# Autodesk Inventor assembly: Assembly1
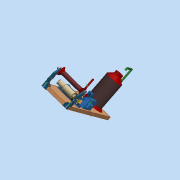
[picture p0: Inventor's stored thumbnail of the model, 180x180]
Saved by Autodesk Inventor 2019 (Build 230136000, 136)
## iProperties
Part Number: Assembly1
Document SubType Name: Assembly
Designer: Dell
Author: Dell
## Documents named in this file (18)
- C:\Users\Dell\Documents\exploration\Assembly1.iam
- C:\Users\Dell\Documents\exploration\base.ipt
- C:\Users\Dell\Documents\exploration\part1.ipt
- C:\Users\Dell\Documents\exploration\part1_MIR.ipt
- C:\Users\Dell\Documents\exploration\part5.ipt
- C:\Users\Dell\Documents\exploration\part3.ipt
- C:\Users\Dell\Documents\exploration\part7.ipt
- C:\Users\Dell\Documents\exploration\spool 2.ipt
- C:\Users\Dell\Documents\Inventor\Content Center Files\R2019\en-US\UNI ISO 1224 M\ISO 1224 - 18 4 x  9 x  2.5.ipt
- C:\Users\Dell\Documents\exploration\spool part.ipt
- C:\Users\Dell\Documents\exploration\spool new.ipt
- C:\Users\Dell\Documents\Inventor\Content Center Files\R2019\en-US\GB 29.2-88\Bolt GB 29.2 M4 x 8.ipt
- C:\Users\Dell\Documents\exploration\hook stand new.ipt
- C:\Users\Dell\Documents\exploration\belt drive part 1.ipt
- C:\Users\Dell\Documents\exploration\dc motor.ipt
- C:\Users\Dell\Documents\exploration\belt drive part 2.ipt
- C:\Users\Dell\Documents\exploration\Part4.ipt
- C:\Users\Dell\Documents\exploration\servo motor.ipt
## Components (21 placed, 17 different names)
1. base:1 — Rotational:1, Rotational:2, Rigid:1, Rigid:2, Rotational:3, Rotational:4, Rigid:6
2. part1:1 — Rotational:1, Cylindrical:1, Rotational:5, Rigid:7
3. part1_MIR:1 — Rotational:2, Rigid:3, Rigid:5
4. part5:1 — Rigid:1, Rigid:9, Rotational:7, Rotational:8
5. part3:1 — Rigid:2
6. part7:1 — Rotational:3
7. spool 2:1 — Rotational:4
8. UNI ISO 1224 (mm) 18 4 x  9 x  2.5:1 — Rigid:3, Rigid:4
9. UNI ISO 1224 (mm) 18 4 x  9 x  2.5:2 — Cylindrical:1
10. spool part:1 — Rigid:4, Cylindrical:2, Rotational:6
11. spool new:1 — Cylindrical:2
12. Bolt GB/T 29.2-1988 M4x8:1 — Rigid:5
13. Bolt GB/T 29.2-1988 M4x8:2 — Rotational:5
14. hook stand new:1 — Rigid:6
15. belt drive part 1:1 — Rotational:6
16. dc motor:1 — Rigid:7, Rigid:8
17. belt drive part 2:1 — Rigid:8
18. Part4:1 — Rigid:10
19. servo motor:1 — Rigid:9, Rigid:10
20. Bolt GB/T 29.2-1988 M4x8:3 — Rotational:7
21. Bolt GB/T 29.2-1988 M4x8:4 — Rotational:8
## Relationships (20: WeldJoint 10, RevoluteJoint 8, CylindricalJoint 2)
- Rotational:1 [RevoluteJoint]: base:1 ↔ part1:1
- Rotational:2 [RevoluteJoint]: base:1 ↔ part1_MIR:1
- Rigid:1 [WeldJoint]: base:1 ↔ part5:1
- Rigid:2 [WeldJoint]: base:1 ↔ part3:1
- Rotational:3 [RevoluteJoint]: base:1 ↔ part7:1
- Rotational:4 [RevoluteJoint]: base:1 ↔ spool 2:1
- Rigid:3 [WeldJoint]: part1_MIR:1 ↔ UNI ISO 1224 (mm) 18 4 x  9 x  2.5:1
- Cylindrical:1: part1:1 ↔ UNI ISO 1224 (mm) 18 4 x  9 x  2.5:2
- Rigid:4 [WeldJoint] (-9 mm): UNI ISO 1224 (mm) 18 4 x  9 x  2.5:1 ↔ spool part:1
- Cylindrical:2: spool part:1 ↔ spool new:1
- Rigid:5 [WeldJoint]: part1_MIR:1 ↔ Bolt GB/T 29.2-1988 M4x8:1
- Rotational:5 [RevoluteJoint]: part1:1 ↔ Bolt GB/T 29.2-1988 M4x8:2
- Rigid:6 [WeldJoint]: base:1 ↔ hook stand new:1
- Rotational:6 [RevoluteJoint]: spool part:1 ↔ belt drive part 1:1
- Rigid:7 [WeldJoint]: part1:1 ↔ dc motor:1
- Rigid:8 [WeldJoint]: dc motor:1 ↔ belt drive part 2:1
- Rigid:9 [WeldJoint]: part5:1 ↔ servo motor:1
- Rigid:10 [WeldJoint]: Part4:1 ↔ servo motor:1
- Rotational:7 [RevoluteJoint]: part5:1 ↔ Bolt GB/T 29.2-1988 M4x8:3
- Rotational:8 [RevoluteJoint]: part5:1 ↔ Bolt GB/T 29.2-1988 M4x8:4
